# Autodesk Inventor assembly: double lift
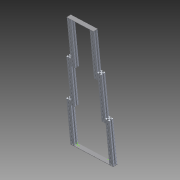
[picture p0: Inventor's stored thumbnail of the model, 180x180]
Saved by Autodesk Inventor 2015 (Build 190159000, 159)
## iProperties
Created: 2014-11-13
Part Number: double lift
Document SubType Name: Assembly
Designer: kruegerma
Mass: 1810.17 g
Surface Area: 8307.86 cm^2
Volume: 1810.17 cm^3
Density: 1 g/cm^3
Author: kruegerma
## Documents named in this file (4)
- E:\double lift.iam
- E:\lift 1.iam
- E:\cross bar.ipt
- E:\Bottom bar.ipt
## Components (4 placed, 3 different names)
1. lift 1:1 [sub-assembly] — Mate:1, Flush:1, Flush:2, Mate:3, Flush:5
2. lift 1:2 [sub-assembly] — Flush:3, Mate:2, Flush:4, Flush:6, Mate:4
3. cross bar:1 — Mate:1, Flush:1, Flush:2, Flush:3, Mate:2, Flush:4
4. Bottom bar:1 — Mate:3, Flush:5, Flush:6, Mate:4
## Relationships (10: Flush 6, Mate 4)
- Mate:1: lift 1:1 ↔ cross bar:1
- Flush:1: lift 1:1 ↔ cross bar:1
- Flush:2: lift 1:1 ↔ cross bar:1
- Flush:3: lift 1:2 ↔ cross bar:1
- Mate:2: lift 1:2 ↔ cross bar:1
- Flush:4: lift 1:2 ↔ cross bar:1
- Mate:3: lift 1:1 ↔ Bottom bar:1
- Flush:5: lift 1:1 ↔ Bottom bar:1
- Flush:6: lift 1:2 ↔ Bottom bar:1
- Mate:4: lift 1:2 ↔ Bottom bar:1
